# Autodesk Inventor assembly: V07-Assembly
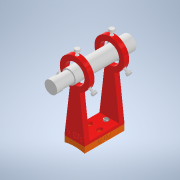
[picture p0: Inventor's stored thumbnail of the model, 180x180]
Saved by Autodesk Inventor 2021.1 (Build 251245000, 245)
## iProperties
Created: 2020-07-26
Part Number: V07-Assembly
Document SubType Name: Assembly
Designer: robst
Author: robst
## Documents named in this file (8)
- C:\git\CAD-Development\robSteele\ShapeWays\TelescopeProjects\CelestronFinderScope\V07-Assembly.iam
- C:\git\CAD-Development\robSteele\ShapeWays\TelescopeProjects\CelestronFinderScope\finderSupportPartV07.ipt
- C:\git\CAD-Development\robSteele\ShapeWays\TelescopeProjects\CelestronFinderScope\finderMainPartV07.ipt
- c:\git\CAD-MfgResources\McMaster-Carr\Insert\10-32x0_310_BRASS HEAT-SET INSERT FOR PLASTIC.ipt
- C:\Users\robst\Documents\Inventor\Content Center Files\R2021\en-US\U UNC 2605\Unbrako - 10 x 1_2 - 32(10).ipt
- c:\git\CAD-MfgResources\McMaster-Carr\Screw\91746A226_18-8 STAINLESS STEEL KNURLED HEAD THUMB SCREW.ipt
- c:\git\CAD-MfgResources\McMaster-Carr\Insert\8-32x0_250_BRASS HEAT-SET INSERT FOR PLASTIC.ipt
- C:\git\CAD-Development\robSteele\ShapeWays\TelescopeProjects\CelestronFinderScope\celestronFinder.ipt
## Components (19 placed, 7 different names)
1. finderSupportPartV07:1 — Insert:1, Insert:2, Insert:3, Flush:1, Flush:2
2. finderMainPartV07:1 — Insert:3, Flush:1, Flush:2, Insert:4, Insert:5, Insert:6, Insert:7, Insert:8, Insert:9, Insert:10, Insert:11, Insert:12, Insert:13, Insert:14, Insert:15, Insert:16, Insert:17, Insert:18
3. 10-32x0_310_BRASS HEAT-SET INSERT FOR PLASTIC:1 — Insert:1
4. 10-32x0_310_BRASS HEAT-SET INSERT FOR PLASTIC:2 — Insert:2
5. Unbrako UNC Hex Socket Button Cap - Inch 10 x 1/2:1 — Insert:4
6. Unbrako UNC Hex Socket Button Cap - Inch 10 x 1/2:2 — Insert:5
7. 91746A226_18-8 STAINLESS STEEL KNURLED HEAD THUMB SCREW:1 — Insert:6
8. 91746A226_18-8 STAINLESS STEEL KNURLED HEAD THUMB SCREW:2 — Insert:7
9. 91746A226_18-8 STAINLESS STEEL KNURLED HEAD THUMB SCREW:3 — Insert:8
10. 91746A226_18-8 STAINLESS STEEL KNURLED HEAD THUMB SCREW:4 — Insert:9
11. 91746A226_18-8 STAINLESS STEEL KNURLED HEAD THUMB SCREW:5 — Insert:11
12. 91746A226_18-8 STAINLESS STEEL KNURLED HEAD THUMB SCREW:6 — Insert:10
13. 8-32x0_250_BRASS HEAT-SET INSERT FOR PLASTIC:1 — Insert:12
14. 8-32x0_250_BRASS HEAT-SET INSERT FOR PLASTIC:2 — Insert:13
15. 8-32x0_250_BRASS HEAT-SET INSERT FOR PLASTIC:3 — Insert:14
16. 8-32x0_250_BRASS HEAT-SET INSERT FOR PLASTIC:4 — Insert:15
17. 8-32x0_250_BRASS HEAT-SET INSERT FOR PLASTIC:5 — Insert:16
18. 8-32x0_250_BRASS HEAT-SET INSERT FOR PLASTIC:6 — Insert:17
19. celestronFinder:1 — Insert:18
## Relationships (20: Insert 18, Flush 2)
- Insert:1: finderSupportPartV07:1 ↔ 10-32x0_310_BRASS HEAT-SET INSERT FOR PLASTIC:1
- Insert:2: finderSupportPartV07:1 ↔ 10-32x0_310_BRASS HEAT-SET INSERT FOR PLASTIC:2
- Insert:3: finderSupportPartV07:1 ↔ finderMainPartV07:1
- Flush:1: finderSupportPartV07:1 ↔ finderMainPartV07:1
- Flush:2: finderSupportPartV07:1 ↔ finderMainPartV07:1
- Insert:4: finderMainPartV07:1 ↔ Unbrako UNC Hex Socket Button Cap - Inch 10 x 1/2:1
- Insert:5: finderMainPartV07:1 ↔ Unbrako UNC Hex Socket Button Cap - Inch 10 x 1/2:2
- Insert:6 (12.7 mm): finderMainPartV07:1 ↔ 91746A226_18-8 STAINLESS STEEL KNURLED HEAD THUMB SCREW:1
- Insert:7 (12.7 mm): finderMainPartV07:1 ↔ 91746A226_18-8 STAINLESS STEEL KNURLED HEAD THUMB SCREW:2
- Insert:8 (12.7 mm): finderMainPartV07:1 ↔ 91746A226_18-8 STAINLESS STEEL KNURLED HEAD THUMB SCREW:3
- Insert:9 (12.7 mm): finderMainPartV07:1 ↔ 91746A226_18-8 STAINLESS STEEL KNURLED HEAD THUMB SCREW:4
- Insert:10 (12.7 mm): finderMainPartV07:1 ↔ 91746A226_18-8 STAINLESS STEEL KNURLED HEAD THUMB SCREW:6
- Insert:11 (12.7 mm): finderMainPartV07:1 ↔ 91746A226_18-8 STAINLESS STEEL KNURLED HEAD THUMB SCREW:5
- Insert:12: finderMainPartV07:1 ↔ 8-32x0_250_BRASS HEAT-SET INSERT FOR PLASTIC:1
- Insert:13: finderMainPartV07:1 ↔ 8-32x0_250_BRASS HEAT-SET INSERT FOR PLASTIC:2
- Insert:14: finderMainPartV07:1 ↔ 8-32x0_250_BRASS HEAT-SET INSERT FOR PLASTIC:3
- Insert:15: finderMainPartV07:1 ↔ 8-32x0_250_BRASS HEAT-SET INSERT FOR PLASTIC:4
- Insert:16: finderMainPartV07:1 ↔ 8-32x0_250_BRASS HEAT-SET INSERT FOR PLASTIC:5
- Insert:17: finderMainPartV07:1 ↔ 8-32x0_250_BRASS HEAT-SET INSERT FOR PLASTIC:6
- Insert:18 (45.72 mm): finderMainPartV07:1 ↔ celestronFinder:1
